# Autodesk Inventor assembly: TelescopingArm_MIR
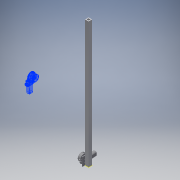
[picture p0: Inventor's stored thumbnail of the model, 180x180]
Saved by Autodesk Inventor 2016 SP1 (Build 200210100, 210)
## iProperties
Created: 2016-01-26
Part Number: TelescopingArm_MIR
Document SubType Name: Assembly
Designer: steele
Author: steele
## Documents named in this file (5)
- C:\snobotics\CAD-Development\robSteele\SnoBotics2016\TelescopeArm\TelescopingArm_MIR.iam
- C:\snobotics\CAD-Development\robSteele\SnoBotics2016\TelescopeArm\1_250_inchSquareTube_MIR.ipt
- C:\snobotics\CAD-Development\robSteele\SnoBotics2016\AM Parts\SnowBlowerMotorAndHub_MIR.iam
- C:\snobotics\CAD-Development\robSteele\SnoBotics2016\TelescopeArm\PlateForConnectionToArm_MIR.ipt
- C:\snobotics\CAD-Development\robSteele\SnoBotics2016\TelescopeArm\1_000_inchSquareTube_MIR.ipt
## Components (4 placed, 4 different names)
1. 1_250_inchSquareTube_MIR:1 — Mate:2, Flush:1, Mate:1, Flush:2, Mate:4, Mate:3
2. SnowBlowerMotorAndHub_MIR:1 [sub-assembly] — Insert:1
3. PlateForConnectionToArm_MIR:1 — Insert:1, Mate:2, Flush:1, Mate:1
4. 1_000_inchSquareTube_MIR:1 — Flush:2, Mate:4, Mate:3
## Relationships (7: Mate 4, Flush 2, Insert 1)
- Insert:1: SnowBlowerMotorAndHub_MIR:1 ↔ PlateForConnectionToArm_MIR:1
- Mate:2: 1_250_inchSquareTube_MIR:1 ↔ PlateForConnectionToArm_MIR:1
- Flush:1: 1_250_inchSquareTube_MIR:1 ↔ PlateForConnectionToArm_MIR:1
- Mate:1: 1_250_inchSquareTube_MIR:1 ↔ PlateForConnectionToArm_MIR:1
- Flush:2: 1_250_inchSquareTube_MIR:1 ↔ 1_000_inchSquareTube_MIR:1
- Mate:4: 1_250_inchSquareTube_MIR:1 ↔ 1_000_inchSquareTube_MIR:1
- Mate:3: 1_250_inchSquareTube_MIR:1 ↔ 1_000_inchSquareTube_MIR:1
